# Autodesk Inventor assembly: Main_Assembly
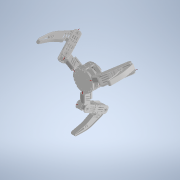
[picture p0: Inventor's stored thumbnail of the model, 180x180]
Saved by Autodesk Inventor 2020.1 (Build 241239000, 239)
## iProperties
Created: 2022-03-07
Part Number: Main_Assembly
Document SubType Name: Assembly
Designer: OEM
Author: OEM
## Documents named in this file (10)
- D:\Studia\Zebulon05\Zebulon05\CAD\Main_Assembly.iam
- D:\Studia\Zebulon05\Zebulon05\CAD\Body.ipt
- D:\Studia\Zebulon05\Zebulon05\CAD\leg0.ipt
- D:\Studia\Zebulon05\Zebulon05\CAD\Servo\HORN-D.ipt
- D:\Studia\Zebulon05\Zebulon05\CAD\Servo\Case.ipt
- D:\Studia\Zebulon05\Zebulon05\CAD\Leg1.ipt
- D:\Studia\Zebulon05\Zebulon05\CAD\RPi Subs.ipt
- D:\Studia\Zebulon05\Zebulon05\CAD\Spacer.ipt
- D:\Studia\Zebulon05\Zebulon05\CAD\Leg2.ipt
- D:\Studia\Zebulon05\Zebulon05\CAD\Leg3.ipt
## Components (43 placed, 14 different names)
1. Bod_lvl_plus1 — Mate:24, Mate:25, Mate:26, Mate:35, Mate:36, Mate:39
2. Body_lvl_Rpi — Mate:15, Mate:16, Mate:17, Mate:21, Mate:22, Mate:23, Mate:27, Mate:28, Mate:29, Mate:34, Mate:38, Mate:41, Mate:44, Mate:45, Mate:46, Mate:47, Mate:131, Mate:132, Mate:133, Mate:134, Mate:135, Mate:136
3. Body_lvl_FPGA — Mate:30, Mate:31, Mate:32, Mate:33, Mate:37, Mate:40, Mate:42, Mate:43
4. leg_part_0 — Mate:15, Mate:16, Mate:17, Mate:48, Mate:49, Mate:50
5. Leg_part_1 — Mate:51, Mate:52, Mate:53, Mate:54, Mate:55, Mate:56
6. Leg_part_3 — Mate:69, Mate:70, Mate:71
7. leg0:2 — Mate:131, Mate:132, Mate:133
8. HORN-D:4
9. Case:7
10. Leg1:2
11. Case:8
12. HORN-D:5
13. Leg2:5
14. Leg2:6
15. HORN-D:6
16. Case:9 — Mate:137, Mate:138, Mate:139
17. Leg3:2 — Mate:137, Mate:138, Mate:139
18. leg0:3 — Mate:134, Mate:135, Mate:136
19. HORN-D:7
20. Case:10
21. Leg1:3
22. Case:11
23. HORN-D:8
24. Leg2:7
25. Leg2:8
26. HORN-D:9
27. Case:12
28. Leg3:3
29. Spacer:8 — Mate:33, Mate:34, Mate:37
30. Spacer:7 — Mate:39, Mate:41, Mate:44
31. Spacer:6 — Mate:35, Mate:36, Mate:38
32. Spacer:5 — Mate:40, Mate:42, Mate:43
33. Spacer:3 — Mate:21, Mate:22, Mate:23, Mate:24, Mate:25, Mate:26
34. Spacer:4 — Mate:27, Mate:28, Mate:29, Mate:30, Mate:31, Mate:32
35. RPi Subs:1 — Mate:45, Mate:46, Mate:47
36. Case:3 — Mate:8, Mate:9, Mate:51, Mate:52, Mate:53
37. HORN-D:1 — Mate:8, Mate:9, Mate:48, Mate:49, Mate:50
38. HORN-D:2 — Mate:13, Mate:14, Mate:58, Mate:59, Mate:60
39. Case:5 — Mate:13, Mate:14, Mate:54, Mate:55, Mate:56, Mate:57
40. Leg2:4 — Mate:61, Mate:62, Mate:63
41. Leg2:2 — Mate:57, Mate:58, Mate:59, Mate:60, Mate:61, Mate:62, Mate:63, Mate:72, Mate:73, Mate:74
42. Case:6 — Mate:67, Mate:68, Mate:69, Mate:70, Mate:71
43. HORN-D:3 — Mate:67, Mate:68, Mate:72, Mate:73, Mate:74
## Relationships (120: Mate 120)
- Mate:8: Case:3 ↔ HORN-D:1
- Mate:9: Case:3 ↔ HORN-D:1
- Mate:13: HORN-D:2 ↔ Case:5
- Mate:14: HORN-D:2 ↔ Case:5
- Mate:15: Body_lvl_Rpi ↔ leg_part_0
- Mate:16: Body_lvl_Rpi ↔ leg_part_0
- Mate:17: Body_lvl_Rpi ↔ leg_part_0
- Mate:21: Body_lvl_Rpi ↔ Spacer:3
- Mate:22: Body_lvl_Rpi ↔ Spacer:3
- Mate:23: Body_lvl_Rpi ↔ Spacer:3
- Mate:24: Bod_lvl_plus1 ↔ Spacer:3
- Mate:25: Bod_lvl_plus1 ↔ Spacer:3
- Mate:26: Bod_lvl_plus1 ↔ Spacer:3
- Mate:27: Body_lvl_Rpi ↔ Spacer:4
- Mate:28: Body_lvl_Rpi ↔ Spacer:4
- Mate:29: Body_lvl_Rpi ↔ Spacer:4
- Mate:30: Body_lvl_FPGA ↔ Spacer:4
- Mate:31: Body_lvl_FPGA ↔ Spacer:4
- Mate:32: Body_lvl_FPGA ↔ Spacer:4
- Mate:33: Body_lvl_FPGA ↔ Spacer:8
- Mate:34: Body_lvl_Rpi ↔ Spacer:8
- Mate:35: Bod_lvl_plus1 ↔ Spacer:6
- Mate:36: Bod_lvl_plus1 ↔ Spacer:6
- Mate:37: Body_lvl_FPGA ↔ Spacer:8
- Mate:38: Body_lvl_Rpi ↔ Spacer:6
- Mate:39: Bod_lvl_plus1 ↔ Spacer:7
- Mate:40: Body_lvl_FPGA ↔ Spacer:5
- Mate:41: Body_lvl_Rpi ↔ Spacer:7
- Mate:42: Body_lvl_FPGA ↔ Spacer:5
- Mate:43: Body_lvl_FPGA ↔ Spacer:5
- Mate:44: Body_lvl_Rpi ↔ Spacer:7
- Mate:45: Body_lvl_Rpi ↔ RPi Subs:1
- Mate:46: Body_lvl_Rpi ↔ RPi Subs:1
- Mate:47: Body_lvl_Rpi ↔ RPi Subs:1
- Mate:48: leg_part_0 ↔ HORN-D:1
- Mate:49: leg_part_0 ↔ HORN-D:1
- Mate:50: leg_part_0 ↔ HORN-D:1
- Mate:51: Leg_part_1 ↔ Case:3
- Mate:52: Leg_part_1 ↔ Case:3
- Mate:53: Leg_part_1 ↔ Case:3
- Mate:54: Leg_part_1 ↔ Case:5
- Mate:55: Leg_part_1 ↔ Case:5
- Mate:56: Leg_part_1 ↔ Case:5
- Mate:57: Case:5 ↔ Leg2:2
- Mate:58: HORN-D:2 ↔ Leg2:2
- Mate:59: HORN-D:2 ↔ Leg2:2
- Mate:60: HORN-D:2 ↔ Leg2:2
- Mate:61: Leg2:4 ↔ Leg2:2
- Mate:62: Leg2:4 ↔ Leg2:2
- Mate:63: Leg2:4 ↔ Leg2:2
- Mate:67: Case:6 ↔ HORN-D:3
- Mate:68: Case:6 ↔ HORN-D:3
- Mate:69: Leg_part_3 ↔ Case:6
- Mate:70: Leg_part_3 ↔ Case:6
- Mate:71: Leg_part_3 ↔ Case:6
- Mate:72: Leg2:2 ↔ HORN-D:3
- Mate:73: Leg2:2 ↔ HORN-D:3
- Mate:74: Leg2:2 ↔ HORN-D:3
- [Mate]: HORN-D:4 ↔ Case:7
- [Mate]: HORN-D:4 ↔ Case:7
- [Mate]: Case:8 ↔ HORN-D:5
- [Mate]: Case:8 ↔ HORN-D:5
- [Mate]: leg0:2 ↔ HORN-D:4
- [Mate]: leg0:2 ↔ HORN-D:4
- [Mate]: leg0:2 ↔ HORN-D:4
- [Mate]: Case:7 ↔ Leg1:2
- [Mate]: Case:7 ↔ Leg1:2
- [Mate]: Case:7 ↔ Leg1:2
- [Mate]: Leg1:2 ↔ Case:8
- [Mate]: Leg1:2 ↔ Case:8
- [Mate]: Leg1:2 ↔ Case:8
- [Mate]: Case:8 ↔ Leg2:5
- [Mate]: HORN-D:5 ↔ Leg2:5
- [Mate]: HORN-D:5 ↔ Leg2:5
- [Mate]: HORN-D:5 ↔ Leg2:5
- [Mate]: Leg2:5 ↔ Leg2:6
- [Mate]: Leg2:5 ↔ Leg2:6
- [Mate]: Leg2:5 ↔ Leg2:6
- [Mate]: HORN-D:6 ↔ Case:9
- [Mate]: HORN-D:6 ↔ Case:9
- [Mate]: Leg2:5 ↔ HORN-D:6
- [Mate]: Leg2:5 ↔ HORN-D:6
- [Mate]: Leg2:5 ↔ HORN-D:6
- [Mate]: HORN-D:7 ↔ Case:10
- [Mate]: HORN-D:7 ↔ Case:10
- [Mate]: Case:11 ↔ HORN-D:8
- [Mate]: Case:11 ↔ HORN-D:8
- [Mate]: leg0:3 ↔ HORN-D:7
- [Mate]: leg0:3 ↔ HORN-D:7
- [Mate]: leg0:3 ↔ HORN-D:7
- [Mate]: Case:10 ↔ Leg1:3
- [Mate]: Case:10 ↔ Leg1:3
- [Mate]: Case:10 ↔ Leg1:3
- [Mate]: Leg1:3 ↔ Case:11
- [Mate]: Leg1:3 ↔ Case:11
- [Mate]: Leg1:3 ↔ Case:11
- [Mate]: Case:11 ↔ Leg2:7
- [Mate]: HORN-D:8 ↔ Leg2:7
- [Mate]: HORN-D:8 ↔ Leg2:7
- [Mate]: HORN-D:8 ↔ Leg2:7
- [Mate]: Leg2:7 ↔ Leg2:8
- [Mate]: Leg2:7 ↔ Leg2:8
- [Mate]: Leg2:7 ↔ Leg2:8
- [Mate]: HORN-D:9 ↔ Case:12
- [Mate]: HORN-D:9 ↔ Case:12
- [Mate]: Case:12 ↔ Leg3:3
- [Mate]: Case:12 ↔ Leg3:3
- [Mate]: Case:12 ↔ Leg3:3
- [Mate]: Leg2:7 ↔ HORN-D:9
- [Mate]: Leg2:7 ↔ HORN-D:9
- [Mate]: Leg2:7 ↔ HORN-D:9
- Mate:131: Body_lvl_Rpi ↔ leg0:2
- Mate:132: Body_lvl_Rpi ↔ leg0:2
- Mate:133: Body_lvl_Rpi ↔ leg0:2
- Mate:134: Body_lvl_Rpi ↔ leg0:3
- Mate:135: Body_lvl_Rpi ↔ leg0:3
- Mate:136: Body_lvl_Rpi ↔ leg0:3
- Mate:137: Case:9 ↔ Leg3:2
- Mate:138: Case:9 ↔ Leg3:2
- Mate:139: Case:9 ↔ Leg3:2
## Named parameters: d102_d94 = 0 mm, d103_d95 = 0 mm, d107_d99 = 0 mm, d108_d100 = 0 mm, d109_d101 = 0 mm, d110_d21 = 0 mm, d111_d68 = 0 mm, d112_d69 = 0 mm, d113_d70 = 0 mm, d114_d71 = 0 mm, d115_d72 = 0 mm, d116_d73 = 0 mm, d117_d74 = 0 mm, d118_d75 = 0 mm, d119_d76 = 0 mm, d120_d79 = 0 mm, d121_d80 = 0 mm, d122_d81 = 0 mm, d123_d82 = 0 mm, d124_d83 = 0 mm, d125_d84 = 0 mm, d126_d85 = 0 mm, d127_d22 = 0 mm, d128_d26 = 0 mm, d129_d27 = 0 mm, d130_d94 = 0 mm, d131_d95 = 0 mm, d132_d96 = 0 mm, d133_d97 = 0 mm, d134_d98 = 0 mm, d135_d99 = 0 mm, d136_d100 = 0 mm, d137_d101 = 0 mm, d138_d21 = 0 mm, d139_d68 = 0 mm, d140_d69 = 0 mm, d141_d70 = 0 mm, d142_d71 = 0 mm, d143_d72 = 0 mm, d144_d73 = 0 mm, d145_d74 = 0 mm, d146_d75 = 0 mm, d147_d76 = 0 mm, d148_d79 = 0 mm, d149_d80 = 0 mm, d150_d81 = 0 mm, d151_d82 = 0 mm, d152_d83 = 0 mm, d153_d84 = 0 mm, d154_d85 = 0 mm, d155_d22 = 0 mm, d156_d26 = 0 mm, d157_d27 = 0 mm
